# Autodesk Inventor assembly: Shooter Assembly v2
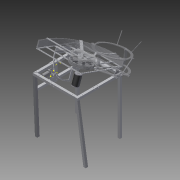
[picture p0: Inventor's stored thumbnail of the model, 180x180]
Saved by Autodesk Inventor 2013 (Build 170138000, 138)
## iProperties
Created: 2013-01-15
Part Number: Shooter Assembly v2
Document SubType Name: Assembly
Designer: actoennies
Mass: 7112.6 g
Surface Area: 21824.2 cm^2
Volume: 3334.32 cm^3
Density: 2.13315 g/cm^3
Author: actoennies
## Documents named in this file (28)
- C:\Users\Moses\Documents\GitHub\frc2013CAD\Launcher\Shooter\Shooter Assembly v2.iam
- C:\Users\Moses\Documents\GitHub\frc2013CAD\Launcher\Shooter\Bearing Mount v1.ipt
- C:\Users\Moses\Documents\GitHub\frc2013CAD\Launcher\Shooter\Outer Rail v1.ipt
- C:\Users\Moses\Documents\GitHub\frc2013CAD\Launcher\Shooter\Runner Rails v2.ipt
- C:\Users\Moses\Documents\GitHub\frc2013CAD\Launcher\Shooter\Bearing.ipt
- C:\Users\Moses\Documents\GitHub\frc2013CAD\Launcher\Shooter\Flywheel Assembly.iam
- C:\Users\Moses\Documents\GitHub\frc2013CAD\Launcher\Shooter\Shooter Mounter.ipt
- C:\Users\Moses\Documents\GitHub\frc2013CAD\Launcher\Shooter\Bearing Mount 2 v1.ipt
- C:\Users\Moses\Documents\GitHub\frc2013CAD\Launcher\Shooter\Shorter Shaft.ipt
- C:\Users\Moses\Documents\GitHub\frc2013CAD\Launcher\Shooter\Spacer Rube.ipt
- C:\Users\Moses\Documents\GitHub\frc2013CAD\Launcher\Shooter\Tower Angled Mount.ipt
- C:\Users\Moses\Documents\GitHub\frc2013CAD\Launcher\Shooter\Edge Mount.ipt
- C:\Users\Moses\Documents\GitHub\frc2013CAD\Launcher\Shooter\Tower Corner Mount.ipt
- C:\Users\Moses\Documents\GitHub\frc2013CAD\Launcher\Shooter\Square Tube.ipt
- C:\Users\Moses\Documents\GitHub\frc2013CAD\Launcher\Shooter\Flange Bearing Mount Tower.ipt
- C:\Users\Moses\Documents\GitHub\frc2013CAD\Launcher\Shooter\Flange Bearing Mount Tower Mirror.ipt
- C:\Users\Moses\Documents\GitHub\frc2013CAD\Launcher\Shooter\Bearing Mount Top.ipt
- C:\Users\Moses\Documents\GitHub\frc2013CAD\Launcher\Shooter\Square Motor Mount.ipt
- C:\Users\Moses\Documents\GitHub\frc2013CAD\Launcher\Hopper\HopperAssembly42inch_v5.iam
- C:\Users\Moses\Documents\GitHub\frc2013CAD\Launcher\Shooter\Shooter Assembly v2\Design Accelerator\Spur Gears1.iam
- C:\Users\Moses\Documents\GitHub\frc2013CAD\Launcher\Parts\Imported Components\Snow Blower Motor\Snow Blower Motor.iam
- C:\Users\Moses\Documents\GitHub\frc2013CAD\Launcher\Shooter\Snowblower Motor Mount.ipt
- C:\Users\Moses\Documents\GitHub\frc2013CAD\Launcher\Shooter\Edge Mount Interference.ipt
- C:\Users\Moses\Documents\GitHub\frc2013CAD\Launcher\Shooter\8mm shaft.ipt
- C:\Users\Moses\Documents\GitHub\frc2013CAD\Launcher\Parts\Imported Components\8mm-key-hub\8mm-key-hub.ipt
- C:\Users\Moses\Documents\GitHub\frc2013CAD\Launcher\Shooter\CIM Bearing.ipt
- C:\Users\Moses\Documents\GitHub\frc2013CAD\Launcher\Parts\CIM Motor\Motors_FR801-001.iam
- C:\Users\Moses\Documents\GitHub\frc2013CAD\Launcher\Parts\8 Plaction Wheel.iam
## Components (37 placed, 27 different names)
1. Bearing Mount v1:1 — Insert:12, Insert:13, Insert:14, Insert:15, Insert:26, Insert:27, Mate:62, Mate:63, Insert:53
2. Outer Rail v1:1 — Insert:12, Insert:13, Insert:47, Insert:48, Flush:21
3. Runner Rails v2:1 — Insert:14, Insert:15, Mate:42, Flush:28
4. Flywheel Assembly:1 [sub-assembly] — Mate:61, Flush:30, Mate:68
5. Shooter Mounter:1 — Insert:26, Insert:27, Insert:34, Flush:11, Insert:35, Insert:36, Insert:37, Insert:38, Flush:19, Mate:45, Flush:24, Angle:3
6. Spacer Rube:1 — Insert:34, Flush:11
7. Bearing Mount 2 v1:1 — Insert:37, Insert:38, Insert:40
8. Bearing Mount 2 v1:2 — Insert:35, Insert:36, Insert:39
9. Bearing:3 — Insert:40, Flush:13, Mate:14, Mate:15
10. Bearing:4 — Insert:39, Flush:12, Mate:12, Mate:13, Mate:36, Mate:44
11. Shorter Shaft:1 — Flush:12, Mate:12, Mate:13, Mate:37
12. Shorter Shaft:2 — Flush:13, Mate:14, Mate:15, Mate:38
13. Tower Angled Mount:1 — Mate:34, Flush:18, Mate:35
14. Tower Corner Mount:1 — Mate:16, Flush:14, Mate:17, Mate:48
15. Edge Mount:2 — Mate:24, Mate:25, Flush:17, Mate:26, Mate:28
16. Square Tube:1 — Mate:21, Mate:33, Mate:34, Flush:18, Mate:49
17. Square Tube:2 — Mate:16, Flush:14, Mate:17, Mate:21, Mate:22, Mate:23, Flush:16, Insert:41, Insert:42, Flush:19, Flush:23, Flush:26, Mate:50, Mate:52, Flush:27
18. Square Tube:3 — Mate:27, Mate:28, Mate:29, Mate:33, Mate:35, Insert:44, Insert:45, Angle:3
19. Square Tube:4 — Mate:22, Mate:23, Flush:16, Mate:24, Mate:25, Flush:17, Mate:26, Mate:27, Mate:29
20. Flange Bearing Mount Tower:1 — Insert:41, Insert:42, Insert:43
21. Bearing:5 — Insert:43, Mate:36, Mate:37
22. Flange Bearing Mount Tower Mirror:1 — Insert:44, Insert:45, Insert:46, Flush:29
23. Bearing:6 — Insert:46, Mate:38
24. Bearing Mount Top:1 — Insert:47, Insert:48, Mate:65, Mate:66, Mate:68
25. Square Motor Mount:1 — Flush:23, Mate:47, Mate:48, Mate:51, Flush:27
26. HopperAssembly42inch_v5:1 [sub-assembly] — Mate:42, Flush:21, Flush:28
27. Spur Gears:1 [sub-assembly] — Mate:44, Mate:45, Flush:24, Flush:25, Mate:46, Angle:2
28. Snow Blower Motor:1 [sub-assembly] — Flush:25, Mate:46, Angle:2, Insert:50, Insert:51
29. Snowblower Motor Mount:1 — Insert:50, Insert:51, Mate:47, Mate:51, Mate:52
30. Edge Mount Interference:1 — Mate:49, Flush:26, Mate:50
31. 8mm shaft:1 — Mate:53, Mate:61, Flush:30, Mate:67, Insert:52
32. 8mm-key-hub:1 — Mate:58, Mate:72, Mate:73
33. 8mm-key-hub:2 — Mate:53, Mate:58, Mate:70, Mate:71, Mate:74, Insert:53
34. CIM Bearing:1 — Mate:65, Mate:66, Mate:67
35. CIM Bearing:2 — Mate:62, Mate:63
36. Motors_FR801-001:1 [sub-assembly] — Insert:52
37. 8 Plaction Wheel:1 [sub-assembly] — Mate:70, Mate:71, Mate:72, Mate:73, Mate:74
## Relationships (89: Mate 45, Insert 25, Flush 17, Angle 2)
- Insert:12: Bearing Mount v1:1 ↔ Outer Rail v1:1
- Insert:13: Bearing Mount v1:1 ↔ Outer Rail v1:1
- Insert:14: Bearing Mount v1:1 ↔ Runner Rails v2:1
- Insert:15: Bearing Mount v1:1 ↔ Runner Rails v2:1
- Insert:26: Bearing Mount v1:1 ↔ Shooter Mounter:1
- Insert:27: Bearing Mount v1:1 ↔ Shooter Mounter:1
- Insert:34: Shooter Mounter:1 ↔ Spacer Rube:1
- Flush:11: Shooter Mounter:1 ↔ Spacer Rube:1
- Insert:35: Shooter Mounter:1 ↔ Bearing Mount 2 v1:2
- Insert:36: Shooter Mounter:1 ↔ Bearing Mount 2 v1:2
- Insert:37: Shooter Mounter:1 ↔ Bearing Mount 2 v1:1
- Insert:38: Shooter Mounter:1 ↔ Bearing Mount 2 v1:1
- Insert:39: Bearing Mount 2 v1:2 ↔ Bearing:4
- Insert:40: Bearing Mount 2 v1:1 ↔ Bearing:3
- Flush:12 (-25.4 mm): Bearing:4 ↔ Shorter Shaft:1
- Mate:12: Bearing:4 ↔ Shorter Shaft:1
- Mate:13: Bearing:4 ↔ Shorter Shaft:1
- Flush:13 (-25.4 mm): Bearing:3 ↔ Shorter Shaft:2
- Mate:14: Bearing:3 ↔ Shorter Shaft:2
- Mate:15: Bearing:3 ↔ Shorter Shaft:2
- Mate:16: Tower Corner Mount:1 ↔ Square Tube:2
- Flush:14: Tower Corner Mount:1 ↔ Square Tube:2
- Mate:17: Tower Corner Mount:1 ↔ Square Tube:2
- Mate:21: Square Tube:1 ↔ Square Tube:2
- Mate:22: Square Tube:2 ↔ Square Tube:4
- Mate:23: Square Tube:2 ↔ Square Tube:4
- Flush:16: Square Tube:2 ↔ Square Tube:4
- Mate:24: Edge Mount:2 ↔ Square Tube:4
- Mate:25: Edge Mount:2 ↔ Square Tube:4
- Flush:17: Edge Mount:2 ↔ Square Tube:4
- Mate:26: Edge Mount:2 ↔ Square Tube:4
- Mate:27: Square Tube:3 ↔ Square Tube:4
- Mate:28: Edge Mount:2 ↔ Square Tube:3
- Mate:29: Square Tube:3 ↔ Square Tube:4
- Mate:33: Square Tube:1 ↔ Square Tube:3
- Mate:34: Tower Angled Mount:1 ↔ Square Tube:1
- Flush:18: Tower Angled Mount:1 ↔ Square Tube:1
- Mate:35: Tower Angled Mount:1 ↔ Square Tube:3
- Insert:41: Square Tube:2 ↔ Flange Bearing Mount Tower:1
- Insert:42: Square Tube:2 ↔ Flange Bearing Mount Tower:1
- Insert:43: Flange Bearing Mount Tower:1 ↔ Bearing:5
- Flush:19: Shooter Mounter:1 ↔ Square Tube:2
- Mate:36: Bearing:4 ↔ Bearing:5
- Mate:37: Shorter Shaft:1 ↔ Bearing:5
- Insert:44: Square Tube:3 ↔ Flange Bearing Mount Tower Mirror:1
- Insert:45: Square Tube:3 ↔ Flange Bearing Mount Tower Mirror:1
- Insert:46: Flange Bearing Mount Tower Mirror:1 ↔ Bearing:6
- Mate:38: Shorter Shaft:2 ↔ Bearing:6
- Insert:47: Outer Rail v1:1 ↔ Bearing Mount Top:1
- Insert:48: Outer Rail v1:1 ↔ Bearing Mount Top:1
- Mate:42: Runner Rails v2:1 ↔ HopperAssembly42inch_v5:1
- Flush:21: Outer Rail v1:1 ↔ HopperAssembly42inch_v5:1
- Flush:23 (152.4 mm): Square Tube:2 ↔ Square Motor Mount:1
- Mate:44: Bearing:4 ↔ Spur Gears:1
- Mate:45 (25.4 mm): Shooter Mounter:1 ↔ Spur Gears:1
- Flush:24: Shooter Mounter:1 ↔ Spur Gears:1
- Flush:25 (-3.175 mm): Spur Gears:1 ↔ Snow Blower Motor:1
- Mate:46: Spur Gears:1 ↔ Snow Blower Motor:1
- Angle:2 (0 deg): Spur Gears:1 ↔ Snow Blower Motor:1
- Insert:50: Snow Blower Motor:1 ↔ Snowblower Motor Mount:1
- Insert:51: Snow Blower Motor:1 ↔ Snowblower Motor Mount:1
- Angle:3 (340 deg): Shooter Mounter:1 ↔ Square Tube:3
- Mate:47: Square Motor Mount:1 ↔ Snowblower Motor Mount:1
- Mate:48: Tower Corner Mount:1 ↔ Square Motor Mount:1
- Mate:49: Square Tube:1 ↔ Edge Mount Interference:1
- Flush:26: Square Tube:2 ↔ Edge Mount Interference:1
- Mate:50: Square Tube:2 ↔ Edge Mount Interference:1
- Mate:51: Square Motor Mount:1 ↔ Snowblower Motor Mount:1
- Mate:52: Square Tube:2 ↔ Snowblower Motor Mount:1
- Flush:27: Square Tube:2 ↔ Square Motor Mount:1
- Flush:28: Runner Rails v2:1 ↔ HopperAssembly42inch_v5:1
- Flush:29 (203.2 mm): Flange Bearing Mount Tower Mirror:1
- Mate:53: 8mm shaft:1 ↔ 8mm-key-hub:2
- Mate:58: 8mm-key-hub:1 ↔ 8mm-key-hub:2
- Mate:61: Flywheel Assembly:1 ↔ 8mm shaft:1
- Flush:30 (6.35 mm): Flywheel Assembly:1 ↔ 8mm shaft:1
- Mate:62: Bearing Mount v1:1 ↔ CIM Bearing:2
- Mate:63: Bearing Mount v1:1 ↔ CIM Bearing:2
- Mate:65: Bearing Mount Top:1 ↔ CIM Bearing:1
- Mate:66: Bearing Mount Top:1 ↔ CIM Bearing:1
- Mate:67: 8mm shaft:1 ↔ CIM Bearing:1
- Mate:68 (6.35 mm): Flywheel Assembly:1 ↔ Bearing Mount Top:1
- Insert:52: 8mm shaft:1 ↔ Motors_FR801-001:1
- Mate:70: 8mm-key-hub:2 ↔ 8 Plaction Wheel:1
- Mate:71: 8mm-key-hub:2 ↔ 8 Plaction Wheel:1
- Mate:72: 8mm-key-hub:1 ↔ 8 Plaction Wheel:1
- Mate:73: 8mm-key-hub:1 ↔ 8 Plaction Wheel:1
- Mate:74: 8mm-key-hub:2 ↔ 8 Plaction Wheel:1
- Insert:53 (6.35 mm): Bearing Mount v1:1 ↔ 8mm-key-hub:2
